# Autodesk Inventor assembly: 5 Barras Version 0
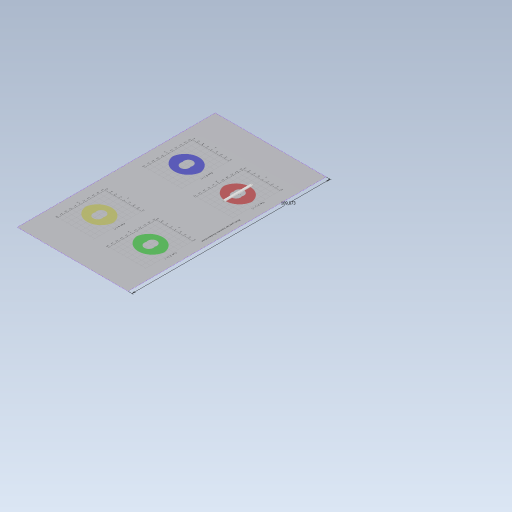
[picture p0: Inventor's stored thumbnail of the model, 512x512]
Saved by Autodesk Inventor 2024.2 (Build 282272000, 272)
## iProperties
Created: 2025-02-06
Part Number: 5 Barras Version 0
Document SubType Name: Assembly
Designer: jp.reyesf
Author: jp.reyesf
## Documents named in this file (18)
- C:\Users\jp.reyesf\Desktop\Master-Thesis\five_bar\assets\CAD\Robot\5 Barras Version 0.iam
- C:\Users\jp.reyesf\Desktop\Master-Thesis\five_bar\assets\CAD\Robot\Proximal Link 1.ipt
- C:\Users\jp.reyesf\Desktop\Master-Thesis\five_bar\assets\CAD\Robot\Distal Link 1.ipt
- C:\Users\jp.reyesf\Desktop\Master-Thesis\five_bar\assets\CAD\Robot\Distal Link 2.ipt
- C:\Users\jp.reyesf\Desktop\Master-Thesis\five_bar\assets\CAD\Robot\Proximal Link 2.ipt
- C:\Users\jp.reyesf\Desktop\Master-Thesis\five_bar\assets\CAD\Robot\Spacer.ipt
- C:\Users\jp.reyesf\Desktop\Master-Thesis\five_bar\assets\CAD\Robot\Bearing.ipt
- C:\Users\jp.reyesf\Desktop\Master-Thesis\five_bar\assets\CAD\Robot\Motor 1 Stator.ipt
- C:\Users\jp.reyesf\Desktop\Master-Thesis\five_bar\assets\CAD\Robot\Motor 1 Rotor.ipt
- C:\Users\jp.reyesf\Desktop\Master-Thesis\five_bar\assets\CAD\Robot\Motor 2 Stator.ipt
- C:\Users\jp.reyesf\Desktop\Master-Thesis\five_bar\assets\CAD\Robot\Motor 2 Rotor.ipt
- C:\Users\jp.reyesf\Desktop\Master-Thesis\five_bar\assets\CAD\Robot\separator.ipt
- C:\Users\jp.reyesf\Desktop\Master-Thesis\five_bar\assets\CAD\Robot\rod.ipt
- C:\Users\jp.reyesf\Desktop\Master-Thesis\five_bar\assets\CAD\Robot\Solid35.ipt
- C:\Users\jp.reyesf\Desktop\Master-Thesis\five_bar\assets\CAD\Robot\Solid37.ipt
- C:\Users\jp.reyesf\Desktop\Master-Thesis\five_bar\assets\CAD\Robot\Solid38.ipt
- C:\Users\jp.reyesf\Desktop\Master-Thesis\five_bar\assets\CAD\Robot\Spacer 2.ipt
- C:\Users\jp.reyesf\Desktop\Master-Thesis\five_bar\assets\CAD\Robot\Solid40.ipt
## Components (37 placed, 17 different names)
1. Proximal Link 1:1 — Mate:3, Mate:4, Mate:5, Mate:39, Mate:91, Mate:92
2. Distal Link 1:1 — Mate:39, Mate:43, Mate:127, Mate:128, Mate:129
3. Distal Link 2:1 — Mate:43, Mate:47, Mate:130, Mate:131, Mate:132
4. Proximal Link 2:1 — Mate:47, Mate:48, Mate:49, Mate:133
5. Motor 1 Stator:1 — Mate:1, Mate:2
6. Motor 1 Rotor:1 — Mate:1, Mate:2, Mate:3, Mate:4, Mate:5
7. Motor 2 Stator:1 — Mate:50, Mate:51
8. Motor 2 Rotor:1 — Mate:48, Mate:49, Mate:50, Mate:51
9. Solid35:1
10. Solid37:1
11. Solid38:1
12. Spacer 2:1
13. Solid40:1
14. separator:2
15. Spacer:5
16. Bearing:14
17. Bearing:15 — Mate:91, Mate:92
18. Bearing:17 — Mate:97, Mate:98
19. rod:2
20. Spacer:7 — Mate:97, Mate:98, Mate:99, Mate:100
21. Bearing:22 — Mate:99, Mate:100, Mate:127
22. separator:3
23. Spacer:8 — Mate:132
24. Bearing:23
25. Bearing:24 — Mate:133
26. Bearing:25
27. rod:3
28. Spacer:9
29. Bearing:26 — Mate:131
30. separator:4
31. Spacer:10
32. Bearing:27 — Mate:129
33. Bearing:28 — Mate:130
34. Bearing:29
35. rod:4
36. Spacer:11
37. Bearing:30 — Mate:128
## Relationships (63: Mate 60, Flush 3)
- Mate:1: Motor 1 Stator:1 ↔ Motor 1 Rotor:1
- Mate:2: Motor 1 Stator:1 ↔ Motor 1 Rotor:1
- Mate:3: Proximal Link 1:1 ↔ Motor 1 Rotor:1
- Mate:4: Proximal Link 1:1 ↔ Motor 1 Rotor:1
- Mate:5: Proximal Link 1:1 ↔ Motor 1 Rotor:1
- Mate:39: Proximal Link 1:1 ↔ Distal Link 1:1
- Mate:43: Distal Link 1:1 ↔ Distal Link 2:1
- Mate:47: Distal Link 2:1 ↔ Proximal Link 2:1
- Mate:48: Proximal Link 2:1 ↔ Motor 2 Rotor:1
- Mate:49: Proximal Link 2:1 ↔ Motor 2 Rotor:1
- Mate:50: Motor 2 Stator:1 ↔ Motor 2 Rotor:1
- Mate:51: Motor 2 Stator:1 ↔ Motor 2 Rotor:1
- [Mate]: Spacer:5 ↔ Bearing:15
- [Mate]: Spacer:5 ↔ Bearing:14
- [Mate] (0.1 mm): separator:2 ↔ Bearing:14
- [Mate] (0.1 mm): separator:2 ↔ Bearing:17
- [Mate]: Spacer:5 ↔ Bearing:15
- [Mate]: Spacer:5 ↔ Bearing:14
- [Mate]: separator:2 ↔ Bearing:14
- [Mate]: separator:2 ↔ Bearing:17
- [Flush]: Bearing:15 ↔ rod:2
- [Mate]: Bearing:15 ↔ rod:2
- Mate:91: Proximal Link 1:1 ↔ Bearing:15
- Mate:92: Proximal Link 1:1 ↔ Bearing:15
- Mate:97: Bearing:17 ↔ Spacer:7
- Mate:98: Bearing:17 ↔ Spacer:7
- Mate:99: Spacer:7 ↔ Bearing:22
- Mate:100: Spacer:7 ↔ Bearing:22
- [Mate]: Spacer:8 ↔ Bearing:24
- [Mate]: Spacer:8 ↔ Bearing:23
- [Mate] (0.1 mm): separator:3 ↔ Bearing:23
- [Mate] (0.1 mm): separator:3 ↔ Bearing:25
- [Mate]: Spacer:8 ↔ Bearing:24
- [Mate]: Spacer:8 ↔ Bearing:23
- [Mate]: separator:3 ↔ Bearing:23
- [Mate]: separator:3 ↔ Bearing:25
- [Flush]: Bearing:24 ↔ rod:3
- [Mate]: Bearing:24 ↔ rod:3
- [Mate]: Bearing:25 ↔ Spacer:9
- [Mate]: Bearing:25 ↔ Spacer:9
- [Mate]: Spacer:9 ↔ Bearing:26
- [Mate]: Spacer:9 ↔ Bearing:26
- [Mate]: Spacer:10 ↔ Bearing:28
- [Mate]: Spacer:10 ↔ Bearing:27
- [Mate] (0.1 mm): separator:4 ↔ Bearing:27
- [Mate] (0.1 mm): separator:4 ↔ Bearing:29
- [Mate]: Spacer:10 ↔ Bearing:28
- [Mate]: Spacer:10 ↔ Bearing:27
- [Mate]: separator:4 ↔ Bearing:27
- [Mate]: separator:4 ↔ Bearing:29
- [Flush]: Bearing:28 ↔ rod:4
- [Mate]: Bearing:28 ↔ rod:4
- [Mate]: Bearing:29 ↔ Spacer:11
- [Mate]: Bearing:29 ↔ Spacer:11
- [Mate]: Spacer:11 ↔ Bearing:30
- [Mate]: Spacer:11 ↔ Bearing:30
- Mate:127: Distal Link 1:1 ↔ Bearing:22
- Mate:128: Distal Link 1:1 ↔ Bearing:30
- Mate:129: Distal Link 1:1 ↔ Bearing:27
- Mate:130: Distal Link 2:1 ↔ Bearing:28
- Mate:131: Distal Link 2:1 ↔ Bearing:26
- Mate:132: Distal Link 2:1 ↔ Spacer:8
- Mate:133: Proximal Link 2:1 ↔ Bearing:24
## Named parameters: d86_d72 = 0 mm, d87_d85 = 0 mm, d88_d73 = 0 mm, d89_d74 = 0.1 mm, d90_d75 = 0.1 mm, d93_d78 = 0 mm, d94_d79 = 0 mm, d95_d80 = 0 mm, d96_d81 = 0 mm, d99_d84 = 0 mm, d127_d123 = 0 mm, d128_d124 = 0 mm, d129_d125 = 0 mm, d130_d126 = 0 mm, d131_d86_d72 = 0 mm, d132_d87_d85 = 0 mm, d133_d88_d73 = 0 mm, d134_d89_d74 = 0.1 mm, d135_d90_d75 = 0.1 mm, d136_d93_d78 = 0 mm, d137_d94_d79 = 0 mm, d138_d95_d80 = 0 mm, d139_d96_d81 = 0 mm, d140_d99_d84 = 0 mm, d141_d123 = 0 mm, d142_d124 = 0 mm, d143_d125 = 0 mm, d144_d126 = 0 mm, d145_d86_d72 = 0 mm, d146_d87_d85 = 0 mm, d147_d88_d73 = 0 mm, d148_d89_d74 = 0.1 mm, d149_d90_d75 = 0.1 mm, d150_d93_d78 = 0 mm, d151_d94_d79 = 0 mm, d152_d95_d80 = 0 mm, d153_d96_d81 = 0 mm, d154_d99_d84 = 0 mm
